# Autodesk Inventor assembly: UQ205-SafeHolder-sample
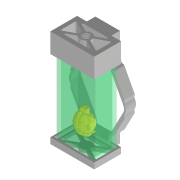
[picture p0: Inventor's stored thumbnail of the model, 180x180]
Saved by Autodesk Inventor 2021 (Build 250183000, 183)
## iProperties
Created: 2023-02-10
Part Number: UQ205-SafeHolder-sample
Document SubType Name: Assembly
Designer: nvladi
Author: nvladi
## Documents named in this file (4)
- C:\Users\Public\GitHub-public\benchtop-hardware\Benchtop\CAD-model-Inventor2021\mesoSPIM\sample_handling\assemblies\UQ205-SafeHolder-sample.iam
- C:\Users\Public\GitHub-public\benchtop-hardware\Benchtop\CAD-model-Inventor2021\library\Portmann Instruments\UQ-205-10x20x45mm.ipt
- C:\Users\Public\GitHub-public\benchtop-hardware\Benchtop\CAD-model-Inventor2021\mesoSPIM\sample_handling\cuvette-holders\Cuvette-22.5x12.5mm(UG205)\Clamp-UG205(204)_100881(1mm Gelenke 2Stk.)_B.ipt
- C:\Users\Public\GitHub-public\benchtop-hardware\Benchtop\CAD-model-Inventor2021\library\samples\mousebrain2.ipt
## Components (3 placed, 3 different names)
1. UQ-205-10x20x45mm:1 — Mate:1, Mate:2, Mate:3
2. Clamp-UG205(204)_100881(1mm Gelenke 2Stk.)_B:1 — Mate:1, Mate:2, Mate:3
3. mousebrain2:1
## Relationships (3: Mate 3)
- Mate:1: UQ-205-10x20x45mm:1 ↔ Clamp-UG205(204)_100881(1mm Gelenke 2Stk.)_B:1
- Mate:2: UQ-205-10x20x45mm:1 ↔ Clamp-UG205(204)_100881(1mm Gelenke 2Stk.)_B:1
- Mate:3 (0.25 mm): UQ-205-10x20x45mm:1 ↔ Clamp-UG205(204)_100881(1mm Gelenke 2Stk.)_B:1
